# Autodesk Inventor assembly: Final asembley button maker
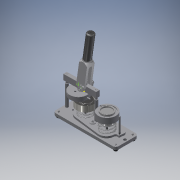
[picture p0: Inventor's stored thumbnail of the model, 180x180]
Saved by Autodesk Inventor 2017.3 (Build 213256000, 256)
## iProperties
Created: 2017-05-01
Part Number: Final asembley button maker
Document SubType Name: Assembly
Designer: rbibb
Author: rbibb
## Documents named in this file (5)
- C:\Users\rbibb\Documents\Enginering\Unit 8\8.1\Final asembley button maker.iam
- C:\Users\rbibb\Documents\Enginering\Unit 8\8.1\Final Assembly Jaden.iam
- C:\Users\rbibb\Documents\Enginering\Unit 8\8.1\Ryan final assembley.iam
- C:\Users\rbibb\Documents\Enginering\Unit 8\8.1\Biblow Asemblee.iam
- C:\Users\rbibb\Documents\Enginering\Unit 8\8.1\jorge's assembly.iam
## Components (4 placed, 4 different names)
1. Final Assembly Jaden:1 [sub-assembly] — Rotational:1, Mate:1, Flush:1
2. Ryan final assembley:1 [sub-assembly] — Rotational:1
3. Biblow Asemblee:1 [sub-assembly] — Rotational:2
4. jorge's assembly:1 [sub-assembly] — Mate:1, Flush:1, Rotational:2
## Relationships (4: RevoluteJoint 2, Mate 1, Flush 1)
- Rotational:1 [RevoluteJoint]: Final Assembly Jaden:1 ↔ Ryan final assembley:1
- Mate:1: Final Assembly Jaden:1 ↔ jorge's assembly:1
- Flush:1: Final Assembly Jaden:1 ↔ jorge's assembly:1
- Rotational:2 [RevoluteJoint]: Biblow Asemblee:1 ↔ jorge's assembly:1
